# Autodesk Inventor assembly: Tray
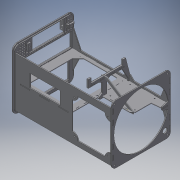
[picture p0: Inventor's stored thumbnail of the model, 180x180]
Saved by Autodesk Inventor 2017 (Build 210142000, 142)
## iProperties
Created: 2019-06-22
Part Number: Tray
Document SubType Name: Assembly
Designer: DDeGo
Author: DDeGo
## Documents named in this file (14)
- C:\Users\DDeGo\OneDrive\Projects\LIT pc case\Tray.iam
- C:\Users\DDeGo\OneDrive\Projects\LIT pc case\TrayPanelA.ipt
- C:\Users\DDeGo\OneDrive\Projects\LIT pc case\TrayPanelB.ipt
- C:\Users\DDeGo\OneDrive\Projects\LIT pc case\TrayPanelC.ipt
- C:\Users\DDeGo\OneDrive\Projects\LIT pc case\TrayPanelD_180mm.ipt
- C:\Users\DDeGo\OneDrive\Projects\LIT pc case\TrayPanelE.ipt
- C:\Users\DDeGo\OneDrive\Projects\LIT pc case\TrayPanelF.ipt
- C:\Users\DDeGo\OneDrive\Projects\LIT pc case\TrayPanelG.ipt
- C:\Users\DDeGo\OneDrive\Projects\LIT pc case\TrayPanelH.ipt
- C:\Users\DDeGo\OneDrive\Projects\LIT pc case\TrayPanelI.ipt
- C:\Users\DDeGo\OneDrive\Projects\LIT pc case\TrayPanelJ.ipt
- C:\Users\DDeGo\OneDrive\Projects\LIT pc case\TrayPanelK.ipt
- C:\Users\DDeGo\OneDrive\Projects\LIT pc case\GPU Clamp.ipt
- C:\Users\DDeGo\OneDrive\Projects\LIT pc case\TrayPanelL.ipt
## Components (13 placed, 13 different names)
1. TrayPanelA:1 — Mate:5, Mate:6, Mate:7, Mate:8, Mate:9, Mate:10, Mate:33
2. TrayPanelB:1 — Mate:1, Flush:1, Flush:2, Mate:18, Mate:19, Mate:20, Mate:21, Mate:22, Mate:23, Mate:27, Mate:28
3. TrayPanelC:1 — Mate:2, Mate:3, Mate:4
4. TrayPanelD_180mm:1 — Flush:3, Flush:4, Mate:11
5. TrayPanelE:1 — Mate:1, Flush:1, Flush:2, Mate:2, Mate:3, Mate:4, Mate:5, Mate:6, Mate:7, Flush:3, Flush:4, Angle:1
6. TrayPanelF:1 — Mate:8, Mate:9, Mate:10, Mate:11, Mate:12, Mate:13, Mate:14
7. TrayPanelG:1 — Mate:12, Mate:13, Mate:14, Mate:15, Mate:16, Mate:17, Mate:32, Mate:34
8. TrayPanelH:1 — Mate:15, Mate:16, Mate:17
9. TrayPanelI:1 — Mate:18, Mate:19, Mate:20, Mate:29, Mate:30, Mate:31
10. TrayPanelJ:1 — Mate:21, Mate:22, Mate:23
11. TrayPanelK:1 — Mate:32, Mate:33, Mate:34
12. GPU Clamp:1 — Mate:27, Mate:28, Angle:1
13. TrayPanelL:1 — Mate:29, Mate:30, Mate:31
## Relationships (36: Mate 31, Flush 4, Angle 1)
- Mate:1: TrayPanelB:1 ↔ TrayPanelE:1
- Flush:1 (3.5 mm): TrayPanelB:1 ↔ TrayPanelE:1
- Flush:2 (3.5 mm): TrayPanelB:1 ↔ TrayPanelE:1
- Mate:2: TrayPanelC:1 ↔ TrayPanelE:1
- Mate:3: TrayPanelC:1 ↔ TrayPanelE:1
- Mate:4: TrayPanelC:1 ↔ TrayPanelE:1
- Mate:5: TrayPanelA:1 ↔ TrayPanelE:1
- Mate:6: TrayPanelA:1 ↔ TrayPanelE:1
- Mate:7: TrayPanelA:1 ↔ TrayPanelE:1
- Mate:8: TrayPanelA:1 ↔ TrayPanelF:1
- Mate:9: TrayPanelA:1 ↔ TrayPanelF:1
- Mate:10: TrayPanelA:1 ↔ TrayPanelF:1
- Flush:3: TrayPanelD_180mm:1 ↔ TrayPanelE:1
- Flush:4: TrayPanelD_180mm:1 ↔ TrayPanelE:1
- Mate:11: TrayPanelD_180mm:1 ↔ TrayPanelF:1
- Mate:12: TrayPanelF:1 ↔ TrayPanelG:1
- Mate:13: TrayPanelF:1 ↔ TrayPanelG:1
- Mate:14: TrayPanelF:1 ↔ TrayPanelG:1
- Mate:15: TrayPanelG:1 ↔ TrayPanelH:1
- Mate:16: TrayPanelG:1 ↔ TrayPanelH:1
- Mate:17: TrayPanelG:1 ↔ TrayPanelH:1
- Mate:18: TrayPanelB:1 ↔ TrayPanelI:1
- Mate:19: TrayPanelB:1 ↔ TrayPanelI:1
- Mate:20: TrayPanelB:1 ↔ TrayPanelI:1
- Mate:21: TrayPanelB:1 ↔ TrayPanelJ:1
- Mate:22: TrayPanelB:1 ↔ TrayPanelJ:1
- Mate:23: TrayPanelB:1 ↔ TrayPanelJ:1
- Mate:27: TrayPanelB:1 ↔ GPU Clamp:1
- Mate:28 (1 mm): TrayPanelB:1 ↔ GPU Clamp:1
- Angle:1 (0 deg): TrayPanelE:1 ↔ GPU Clamp:1
- Mate:29: TrayPanelI:1 ↔ TrayPanelL:1
- Mate:30: TrayPanelI:1 ↔ TrayPanelL:1
- Mate:31: TrayPanelI:1 ↔ TrayPanelL:1
- Mate:32: TrayPanelG:1 ↔ TrayPanelK:1
- Mate:33: TrayPanelA:1 ↔ TrayPanelK:1
- Mate:34: TrayPanelG:1 ↔ TrayPanelK:1
